# Autodesk Inventor assembly: Lifting
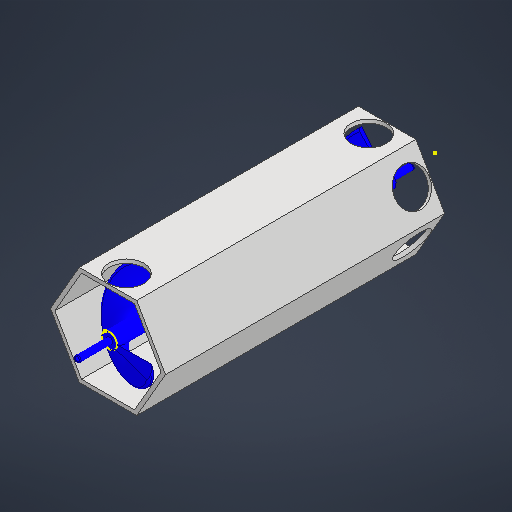
[picture p0: Inventor's stored thumbnail of the model, 512x512]
Saved by Autodesk Inventor 2026.1 (Build 301233020, 233B)
## iProperties
Created: 2026-04-20
Part Number: Lifting
Document SubType Name: Assembly
Designer: hp
Mass: 1144.11 g
Surface Area: 4388.16 cm^2
Volume: 1144.11 cm^3
Density: 1 g/cm^3
Author: hp
## Documents named in this file (4)
- C:\Users\hp\OneDrive\Documents\Inventor\BOM\Lifting.iam
- C:\Users\hp\AppData\Local\Packages\5319275A.WhatsAppDesktop_cv1g1gvanyjgm\LocalState\sessions\53B2033B4B841F2E611008FF6FFFE7CD75AE83E4\transfers\2026-18\hexagon head.ipt
- C:\Users\hp\OneDrive\Documents\Inventor\BOM\hexagon.ipt
- C:\Users\hp\OneDrive\Documents\Inventor\BOM\rod.ipt
## Components (3 placed, 3 different names)
1. rod:1 — Mate:3, Mate:4
2. hexagon head:2 — Mate:3, Mate:4, Mate:7, Mate:8
3. hexagon:1 — Mate:7, Mate:8
## Relationships (4: Mate 4)
- Mate:3: rod:1 ↔ hexagon head:2
- Mate:4 (2 mm): rod:1 ↔ hexagon head:2
- Mate:7: hexagon head:2 ↔ hexagon:1
- Mate:8: hexagon head:2 ↔ hexagon:1
